# Autodesk Inventor assembly: Cockpit_carrier_board_frame
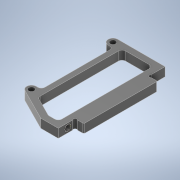
[picture p0: Inventor's stored thumbnail of the model, 180x180]
Saved by Autodesk Inventor 2022.3 (Build 263350000, 350)
## iProperties
Created: 2023-05-14
Part Number: Cockpit_carrier_board_frame
Document SubType Name: Assembly
Designer: Masato Kubotera
Author: Masato Kubotera
## Documents named in this file (3)
- C:\Users\Masato\Documents\Inventor\Inventor for CIT Brains\SUSTAINA-OP - Cockpit mate\UpperBody\Cockpit\Cockpit_carrier_board_frame.iam
- C:\Users\Masato\Documents\Inventor\Inventor for CIT Brains\SUSTAINA-OP - Cockpit mate\UpperBody\Cockpit\Cockpit_carrier_board_frame.ipt
- C:\Users\Masato\Documents\Inventor\Inventor for CIT Brains\SUSTAINA-OP - Cockpit mate\ReadyMade\InsertNut\IRU-304S.ipt
## Components (2 placed, 2 different names)
1. Cockpit_carrier_board_frame:1 — フラッシュ:1, フラッシュ:2, フラッシュ:3, 挿入:1
2. IRU-304S:1 — 挿入:1
## Relationships (4: Flush 3, Insert 1)
- フラッシュ:1 [Flush]: Cockpit_carrier_board_frame:1
- フラッシュ:2 [Flush]: Cockpit_carrier_board_frame:1
- フラッシュ:3 [Flush]: Cockpit_carrier_board_frame:1
- 挿入:1 [Insert]: Cockpit_carrier_board_frame:1 ↔ IRU-304S:1
